# Autodesk Inventor assembly: Сборка1
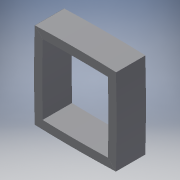
[picture p0: Inventor's stored thumbnail of the model, 180x180]
Saved by Autodesk Inventor 2019 (Build 230136000, 136)
## iProperties
Created: 2019-05-01
Part Number: Сборка1
Material: Типовые
Document SubType Name: Assembly
Designer: stepa
Author: stepa
## Documents named in this file (3)
- C:\Users\stepa\Documents\Inventor\Shamisen\Сборка1.iam
- C:\Users\stepa\Documents\Inventor\Shamisen\Long.ipt
- C:\Users\stepa\Documents\Inventor\Shamisen\Short.ipt
## Components (4 placed, 2 different names)
1. Long:1 — Совмещение:1, Заподлицо:2, Совмещение:4, Заподлицо:3, Заподлицо:4
2. Long:2 — Совмещение:2, Заподлицо:1, Совмещение:3, Заподлицо:5, Заподлицо:6, Совмещение:5
3. Short:1 — Совмещение:2, Заподлицо:1, Совмещение:4, Заподлицо:3, Заподлицо:6, Совмещение:5
4. Short:2 — Совмещение:1, Заподлицо:2, Совмещение:3, Заподлицо:4, Заподлицо:5
## Relationships (11: Flush 6, Mate 5)
- Совмещение:1 [Mate]: Long:1 ↔ Short:2
- Совмещение:2 [Mate]: Long:2 ↔ Short:1
- Заподлицо:1 [Flush]: Long:2 ↔ Short:1
- Заподлицо:2 [Flush]: Long:1 ↔ Short:2
- Совмещение:3 [Mate]: Long:2 ↔ Short:2
- Совмещение:4 [Mate]: Long:1 ↔ Short:1
- Заподлицо:3 [Flush]: Long:1 ↔ Short:1
- Заподлицо:4 [Flush]: Long:1 ↔ Short:2
- Заподлицо:5 [Flush]: Long:2 ↔ Short:2
- Заподлицо:6 [Flush]: Long:2 ↔ Short:1
- Совмещение:5 [Mate]: Long:2 ↔ Short:1
